# Autodesk Inventor assembly: bearing_flat_w_hardware_offset_mirrored
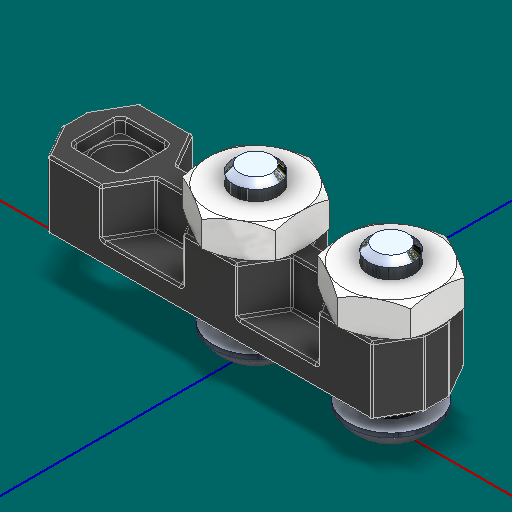
[picture p0: Inventor's stored thumbnail of the model, 512x512]
Saved by Autodesk Inventor 2025 (Build 290162000, 162)
## iProperties
Created: 2024-08-16
Part Number: bearing_flat_w_hardware_offset_mirrored
Document SubType Name: Assembly
Designer: averey
Author: averey
## Documents named in this file (6)
- C:\Users\avere\vex_robotics_high_stakes\hardware\cad\ATLAS\intake\first_stage\arm\arm_half_mirrored\bearing_flat_w_hardware_offset_mirrored.iam
- C:\Users\avere\vex_robotics_high_stakes\hardware\cad\ATLAS\intake\first_stage\arm\arm_half_mirrored\Bearing Flat Low Profile_mirrored.ipt
- C:\Users\avere\vex_robotics_high_stakes\hardware\cad\VEX-CAD-Inventor\Structure\Hardware\Screw Shoulder Robosource\SScrew Shoulder Smooth .500 x .04.ipt
- C:\Users\avere\vex_robotics_high_stakes\hardware\cad\VEX-CAD-Inventor\Structure\Hardware\Screw Shoulder Robosource.ipt
- C:\Users\avere\vex_robotics_high_stakes\hardware\cad\VEX-CAD-Inventor\Structure\Hardware\Nut Nylon\Nut Nylon - White.ipt
- C:\Users\avere\vex_robotics_high_stakes\hardware\cad\VEX-CAD-Inventor\Structure\Hardware\Nut Nylon.ipt
## Components (5 placed, 3 different names)
1. Bearing Flat Low Profile_mirrored:1 — Insert:4, Insert:2, Insert:3
2. SScrew Shoulder Smooth .500 x .04:1 — Insert:4, Mate:1
3. SScrew Shoulder Smooth .500 x .04:2 — Insert:2
4. Nut Nylon - White:1 — Mate:1, Flush:1
5. Nut Nylon - White:2 — Flush:1, Insert:3
## Relationships (5: Insert 3, Mate 1, Flush 1)
- Insert:4 (1.5875 mm): Bearing Flat Low Profile_mirrored:1 ↔ SScrew Shoulder Smooth .500 x .04:1
- Insert:2 (1.5875 mm): Bearing Flat Low Profile_mirrored:1 ↔ SScrew Shoulder Smooth .500 x .04:2
- Mate:1: SScrew Shoulder Smooth .500 x .04:1 ↔ Nut Nylon - White:1
- Flush:1: Nut Nylon - White:1 ↔ Nut Nylon - White:2
- Insert:3 (1.27 mm): Bearing Flat Low Profile_mirrored:1 ↔ Nut Nylon - White:2
